# Autodesk Inventor assembly: outake1.0
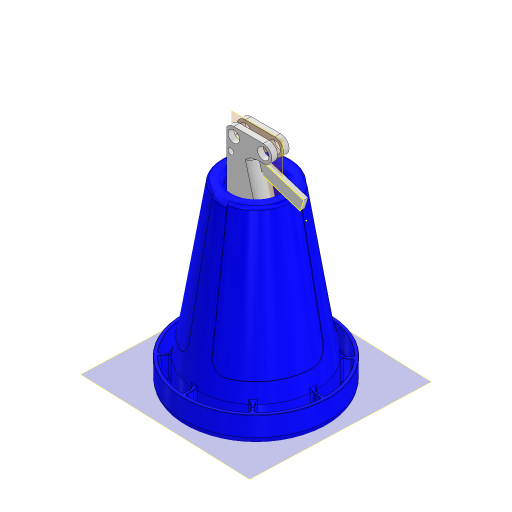
[picture p0: Inventor's stored thumbnail of the model, 512x512]
Saved by Autodesk Inventor 2023 (Build 270158000, 158)
## iProperties
Created: 2022-10-23
Part Number: outake1.0
Document SubType Name: Assembly
Designer: deli
Author: deli
## Documents named in this file (4)
- C:\Users\deli\OneDrive - Eastside Preparatory School\FTC\8103-power-play\CAD\outake1.0.iam
- C:\Users\deli\OneDrive - Eastside Preparatory School\FTC\8103-power-play\CAD\3dPrinting\wedge.ipt
- C:\Users\deli\OneDrive - Eastside Preparatory School\FTC\8103-power-play\CAD\FTC-parts\am-4801_Blue am-4801_Red Cone REV2.ipt
- C:\Users\deli\OneDrive - Eastside Preparatory School\FTC\8103-power-play\CAD\Lever.ipt
## Components (3 placed, 3 different names)
1. wedge:1 — Mate:1, Mate:2, Mate:3
2. am-4801_Blue am-4801_Red Cone REV2:1 — Mate:3, Mate:4
3. Lever:1 — Mate:1, Mate:2, Mate:4
## Relationships (4: Mate 4)
- Mate:1 (0.4125 mm): wedge:1 ↔ Lever:1
- Mate:2: wedge:1 ↔ Lever:1
- Mate:3: wedge:1 ↔ am-4801_Blue am-4801_Red Cone REV2:1
- Mate:4: am-4801_Blue am-4801_Red Cone REV2:1 ↔ Lever:1
